# Autodesk Inventor assembly: KR6-2
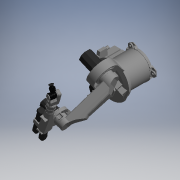
[picture p0: Inventor's stored thumbnail of the model, 180x180]
Saved by Autodesk Inventor 2017 (Build 210142000, 142)
## iProperties
Created: 2015-02-24
Part Number: KR6-2
Document SubType Name: Baugruppe
Designer: Pietro
Manufacturer: Standard
Standards Organization: Custom
Mass: 115449 g
Surface Area: 39949.6 cm^2
Volume: 115449 cm^3
Density: 1 g/cm^3
Übersetzungsnorm: STEP AP214DIS
Dateiname: KR6-2
Vorprozessor: UNIGRAPHICS SOLUTIONS - UNIGRAPHICS 17.0
Postprozessor: Build: 284c, AIS Release: 7 SP1 - Date: Fri 06/06/2003
Gesendete Einheiten: MILLIMETERS
Unbestimmtheit: 0.0
Mass: 115,4 kg
Author: Pietro
## Documents named in this file (14)
- F:\kuka-kr6-1.snapshot.5\KR6.iam
- F:\kuka-kr6-1.snapshot.5\KR6-2 Sockel.ipt
- F:\kuka-kr6-1.snapshot.5\KR6-2 Achse5.ipt
- F:\kuka-kr6-1.snapshot.5\KR6-2 Motor1.ipt
- F:\kuka-kr6-1.snapshot.5\KR6-2 Motor2.ipt
- F:\kuka-kr6-1.snapshot.5\KR6-2 Motor3.ipt
- F:\kuka-kr6-1.snapshot.5\KR6-2 Achse 3.ipt
- F:\kuka-kr6-1.snapshot.5\KR6-2 Achse 6.ipt
- F:\kuka-kr6-1.snapshot.5\KR6-2 Motor4.ipt
- F:\kuka-kr6-1.snapshot.5\KR6-2 Motor5.ipt
- F:\kuka-kr6-1.snapshot.5\KR6-2 Motor6.ipt
- F:\kuka-kr6-1.snapshot.5\KR6-2 Flansch.ipt
- F:\kuka-kr6-1.snapshot.5\KR6-2 Achse 1.ipt
- F:\kuka-kr6-1.snapshot.5\KR6-2 Arm1.ipt
## Components (13 placed, 13 different names)
1. KR6-2 Sockel — Passend:1, Passend:2
2. KR6-2 Achse5 — Passend:10, Passend:11, Passend:14, Passend:18
3. KR6-2 Motor1 — Passend:15, Fluchtend:7, Fluchtend:8
4. KR6-2 Motor2 — Passend:17, Fluchtend:11, Fluchtend:12
5. KR6-2 Motor3 — Passend:16, Fluchtend:9, Fluchtend:10
6. KR6-2 Achse 3 — Passend:5, Fluchtend:1, Fluchtend:2, Passend:6, Passend:7, Passend:8, Fluchtend:3, Fluchtend:4, Passend:9, Fluchtend:5, Fluchtend:6, Passend:10, Passend:11, Passend:15, Fluchtend:7, Fluchtend:8
7. KR6-2 Achse 6 — Passend:12, Passend:13, Passend:14, Passend:18
8. KR6-2 Motor4 — Passend:9, Fluchtend:5, Fluchtend:6
9. KR6-2 Motor5 — Passend:8, Fluchtend:3, Fluchtend:4
10. KR6-2 Motor6 — Passend:5, Fluchtend:1, Fluchtend:2
11. KR6-2 Flansch — Passend:12, Passend:13
12. KR6-2 Achse 1 — Passend:1, Passend:2, Passend:3, Passend:4, Passend:16, Fluchtend:9, Fluchtend:10, Passend:17, Fluchtend:11, Fluchtend:12
13. KR6-2 Arm1 — Passend:3, Passend:4, Passend:6, Passend:7
## Relationships (30: Mate 18, Flush 12)
- Passend:1 [Mate]: KR6-2 Sockel ↔ KR6-2 Achse 1
- Passend:2 [Mate]: KR6-2 Sockel ↔ KR6-2 Achse 1
- Passend:3 [Mate]: KR6-2 Achse 1 ↔ KR6-2 Arm1
- Passend:4 [Mate]: KR6-2 Achse 1 ↔ KR6-2 Arm1
- Passend:5 [Mate]: KR6-2 Achse 3 ↔ KR6-2 Motor6
- Fluchtend:1 [Flush]: KR6-2 Achse 3 ↔ KR6-2 Motor6
- Fluchtend:2 [Flush]: KR6-2 Achse 3 ↔ KR6-2 Motor6
- Passend:6 [Mate]: KR6-2 Achse 3 ↔ KR6-2 Arm1
- Passend:7 [Mate]: KR6-2 Achse 3 ↔ KR6-2 Arm1
- Passend:8 [Mate]: KR6-2 Achse 3 ↔ KR6-2 Motor5
- Fluchtend:3 [Flush]: KR6-2 Achse 3 ↔ KR6-2 Motor5
- Fluchtend:4 [Flush]: KR6-2 Achse 3 ↔ KR6-2 Motor5
- Passend:9 [Mate]: KR6-2 Achse 3 ↔ KR6-2 Motor4
- Fluchtend:5 [Flush]: KR6-2 Achse 3 ↔ KR6-2 Motor4
- Fluchtend:6 [Flush]: KR6-2 Achse 3 ↔ KR6-2 Motor4
- Passend:10 [Mate]: KR6-2 Achse5 ↔ KR6-2 Achse 3
- Passend:11 [Mate]: KR6-2 Achse5 ↔ KR6-2 Achse 3
- Passend:12 [Mate]: KR6-2 Achse 6 ↔ KR6-2 Flansch
- Passend:13 [Mate]: KR6-2 Achse 6 ↔ KR6-2 Flansch
- Passend:14 [Mate]: KR6-2 Achse5 ↔ KR6-2 Achse 6
- Passend:15 [Mate]: KR6-2 Motor1 ↔ KR6-2 Achse 3
- Fluchtend:7 [Flush]: KR6-2 Motor1 ↔ KR6-2 Achse 3
- Fluchtend:8 [Flush]: KR6-2 Motor1 ↔ KR6-2 Achse 3
- Passend:16 [Mate]: KR6-2 Motor3 ↔ KR6-2 Achse 1
- Fluchtend:9 [Flush]: KR6-2 Motor3 ↔ KR6-2 Achse 1
- Fluchtend:10 [Flush]: KR6-2 Motor3 ↔ KR6-2 Achse 1
- Passend:17 [Mate]: KR6-2 Motor2 ↔ KR6-2 Achse 1
- Fluchtend:11 [Flush]: KR6-2 Motor2 ↔ KR6-2 Achse 1
- Fluchtend:12 [Flush]: KR6-2 Motor2 ↔ KR6-2 Achse 1
- Passend:18 [Mate]: KR6-2 Achse5 ↔ KR6-2 Achse 6
